# Autodesk Inventor assembly: RB12
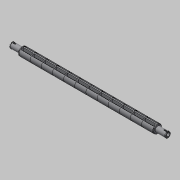
[picture p0: Inventor's stored thumbnail of the model, 180x180]
Saved by Autodesk Inventor 2020 (Build 240168000, 168)
## iProperties
Created: 2019-02-05
Part Number: RB12
Document SubType Name: Assembly
Designer: Varga Daniel
Author: Varga Daniel
## Documents named in this file (5)
- C:\!_Dani\!_cloud\OneDrive\!_munka\Revolution\StructuralParts\Beams\Round beams\RB1+\RB12.iam
- C:\!_Dani\!_cloud\OneDrive\!_munka\Revolution\StructuralParts\Beams\Round Beams\Round_beam_body.ipt
- C:\!_Dani\!_cloud\OneDrive\!_munka\Revolution\StructuralParts\Connector pins\Connector_pin_base.ipt
- C:\!_Dani\!_cloud\OneDrive\!_munka\Revolution\StructuralParts\Connector pins\Connector_pin_base\Connector_pin_base_single_no_anti_skid.ipt
- C:\!_Dani\!_cloud\OneDrive\!_munka\Revolution\StructuralParts\Beams\Round beams\RB1+.iam
## Components (14 placed, 2 different names)
1. Connector_pin_base_single_no_anti_skid:1 — Mate:1, Mate:2, Flush:1
2. Connector_pin_base_single_no_anti_skid:2 — Flush:4, Mate:4, Mate:5
3. Round_beam_body:2 — Flush:2, Flush:3, Mate:3
4. Round_beam_body:3
5. Round_beam_body:4
6. Round_beam_body:5
7. Round_beam_body:6
8. Round_beam_body:7
9. Round_beam_body:8
10. Round_beam_body:9
11. Round_beam_body:10
12. Round_beam_body:11
13. Round_beam_body:12
14. Round_beam_body:13
## Component patterns: (12 elements, first: Round_beam_body:2)
## Relationships (9: Mate 5, Flush 4)
- Mate:1: Connector_pin_base_single_no_anti_skid:1
- Mate:2: Connector_pin_base_single_no_anti_skid:1
- Flush:1: Connector_pin_base_single_no_anti_skid:1
- Flush:2: Round_beam_body:2
- Flush:3: Round_beam_body:2
- Mate:3: Round_beam_body:2
- Flush:4 (-120 mm): Connector_pin_base_single_no_anti_skid:2
- Mate:4: Connector_pin_base_single_no_anti_skid:2
- Mate:5: Connector_pin_base_single_no_anti_skid:2
